# Autodesk Inventor assembly: 42146-16
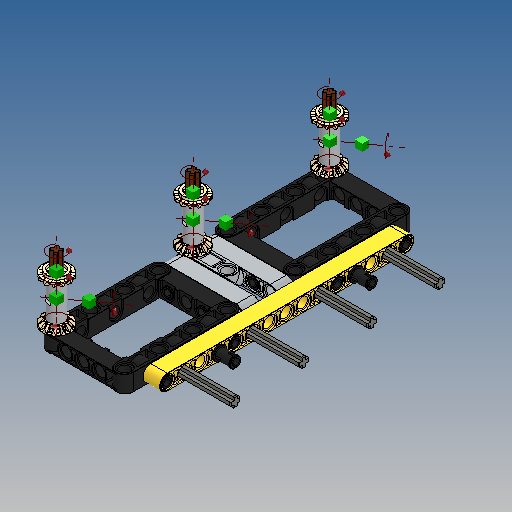
[picture p0: Inventor's stored thumbnail of the model, 512x512]
Saved by Autodesk Inventor 2025 (Build 290162010, 162A)
## iProperties
Created: 2024-11-18
Part Number: 42146-16
Material: Generisch
Document SubType Name: Assembly
Designer: hp.muther
Author: hp.muther
## Documents named in this file (10)
- D:\Inventor\Projekte\Muther\LEGO Technic\LEGO Technik - Raupenkran LR 13000 (42146)\42146-01-16.iam
- D:\Inventor\Projekte\Muther\LEGO Technic\LEGO Pieces\Verbindungselemente\48989-LtBluishGray.ipt
- D:\Inventor\Projekte\Muther\LEGO Technic\LEGO Pieces\Lochbalken\32316-LtBluishGray.ipt
- D:\Inventor\Projekte\Muther\LEGO Technic\LEGO Pieces\Pin's\2780-Black.ipt
- D:\Inventor\Projekte\Muther\LEGO Technic\LEGO Pieces\Rahmen, T-Stücke\64179-Black.ipt
- D:\Inventor\Projekte\Muther\LEGO Technic\LEGO Pieces\Zahnrad\6589-Tan.ipt
- D:\Inventor\Projekte\Muther\LEGO Technic\LEGO Pieces\Rund\62462-LtBluishGray.ipt
- D:\Inventor\Projekte\Muther\LEGO Technic\LEGO Pieces\Achsen\15462-ReddishBrown.ipt
- D:\Inventor\Projekte\Muther\LEGO Technic\LEGO Pieces\Lochbalken\32278-Yellow.ipt
- D:\Inventor\Projekte\Muther\LEGO Technic\LEGO Pieces\Achsen\87083-DkBluishGray.ipt
## Components (32 placed, 9 different names)
1. 48989-LtBluishGray:1 — Einfügen:3, Passend:1, Einfügen:12, Passend:4, Einfügen:16
2. 32316-LtBluishGray:1 — Einfügen:1, Einfügen:2, Einfügen:3, Passend:1, Einfügen:4
3. 2780-Black:1 — Einfügen:5
4. 2780-Black:2 — Einfügen:6
5. 2780-Black:3 — Einfügen:1, Passend:2
6. 2780-Black:4 — Einfügen:2
7. 64179-Black:1 — Einfügen:4, Passend:2, Einfügen:5, Einfügen:6, Einfügen:23, Einfügen:29
8. 32316-LtBluishGray:2 — Einfügen:12, Passend:4
9. 2780-Black:5
10. 2780-Black:6 — Passend:5
11. 2780-Black:7
12. 2780-Black:8
13. 64179-Black:2 — Einfügen:24
14. 6589-Tan:1
15. 6589-Tan:2
16. 62462-LtBluishGray:1
17. 15462-ReddishBrown:1 — Einfügen:16
18. 6589-Tan:3
19. 6589-Tan:4
20. 62462-LtBluishGray:2
21. 15462-ReddishBrown:2 — Einfügen:23
22. 6589-Tan:5
23. 6589-Tan:6
24. 62462-LtBluishGray:3
25. 15462-ReddishBrown:3 — Einfügen:24
26. 32278-Yellow:1 — Einfügen:25, Einfügen:26, Einfügen:27, Einfügen:28, Einfügen:29, Passend:5, Einfügen:30, Einfügen:31
27. 2780-Black:9 — Einfügen:30
28. 2780-Black:10 — Einfügen:31
29. 87083-DkBluishGray:1 — Einfügen:26
30. 87083-DkBluishGray:2 — Einfügen:28
31. 87083-DkBluishGray:3 — Einfügen:27
32. 87083-DkBluishGray:4 — Einfügen:25
## Relationships (36: Insert 31, Mate 5)
- Einfügen:1 [Insert]: 32316-LtBluishGray:1 ↔ 2780-Black:3
- Einfügen:2 [Insert]: 32316-LtBluishGray:1 ↔ 2780-Black:4
- Einfügen:3 [Insert]: 48989-LtBluishGray:1 ↔ 32316-LtBluishGray:1
- Passend:1 [Mate]: 48989-LtBluishGray:1 ↔ 32316-LtBluishGray:1
- Einfügen:4 [Insert]: 32316-LtBluishGray:1 ↔ 64179-Black:1
- Passend:2 [Mate]: 2780-Black:3 ↔ 64179-Black:1
- Einfügen:5 [Insert]: 2780-Black:1 ↔ 64179-Black:1
- Einfügen:6 [Insert]: 2780-Black:2 ↔ 64179-Black:1
- [Insert]: 32316-LtBluishGray:2 ↔ 2780-Black:7
- [Insert]: 32316-LtBluishGray:2 ↔ 2780-Black:8
- [Insert]: 32316-LtBluishGray:2 ↔ 64179-Black:2
- [Mate]: 2780-Black:7 ↔ 64179-Black:2
- [Insert]: 2780-Black:5 ↔ 64179-Black:2
- [Insert]: 2780-Black:6 ↔ 64179-Black:2
- Einfügen:12 [Insert]: 48989-LtBluishGray:1 ↔ 32316-LtBluishGray:2
- Passend:4 [Mate]: 48989-LtBluishGray:1 ↔ 32316-LtBluishGray:2
- [Insert] (7.2 mm): 6589-Tan:1 ↔ 15462-ReddishBrown:1
- [Insert]: 6589-Tan:1 ↔ 62462-LtBluishGray:1
- [Insert]: 6589-Tan:2 ↔ 62462-LtBluishGray:1
- Einfügen:16 [Insert]: 48989-LtBluishGray:1 ↔ 15462-ReddishBrown:1
- [Insert] (7.2 mm): 6589-Tan:3 ↔ 15462-ReddishBrown:2
- [Insert]: 6589-Tan:3 ↔ 62462-LtBluishGray:2
- [Insert]: 6589-Tan:4 ↔ 62462-LtBluishGray:2
- [Insert] (7.2 mm): 6589-Tan:5 ↔ 15462-ReddishBrown:3
- [Insert]: 6589-Tan:5 ↔ 62462-LtBluishGray:3
- [Insert]: 6589-Tan:6 ↔ 62462-LtBluishGray:3
- Einfügen:23 [Insert]: 64179-Black:1 ↔ 15462-ReddishBrown:2
- Einfügen:24 [Insert]: 64179-Black:2 ↔ 15462-ReddishBrown:3
- Einfügen:25 [Insert]: 32278-Yellow:1 ↔ 87083-DkBluishGray:4
- Einfügen:26 [Insert]: 32278-Yellow:1 ↔ 87083-DkBluishGray:1
- Einfügen:27 [Insert]: 32278-Yellow:1 ↔ 87083-DkBluishGray:3
- Einfügen:28 [Insert]: 32278-Yellow:1 ↔ 87083-DkBluishGray:2
- Einfügen:29 [Insert]: 64179-Black:1 ↔ 32278-Yellow:1
- Passend:5 [Mate]: 2780-Black:6 ↔ 32278-Yellow:1
- Einfügen:30 [Insert]: 32278-Yellow:1 ↔ 2780-Black:9
- Einfügen:31 [Insert]: 32278-Yellow:1 ↔ 2780-Black:10
## Named parameters: d8_d0 = 0 mm, d9_d1 = 0 mm, d10_d4 = 0 mm, d11_d5 = 0 mm, d12_d6 = 0 mm, d13_d7 = 0 mm, d20_d179 = 0 mm, d21_d177 = 7.2 mm, d22_d178 = 0 mm, d23_d179 = 0 mm, d24_d177 = 7.2 mm, d25_d178 = 0 mm
